# Autodesk Inventor assembly: mg996r_right_mid_top_two_servo
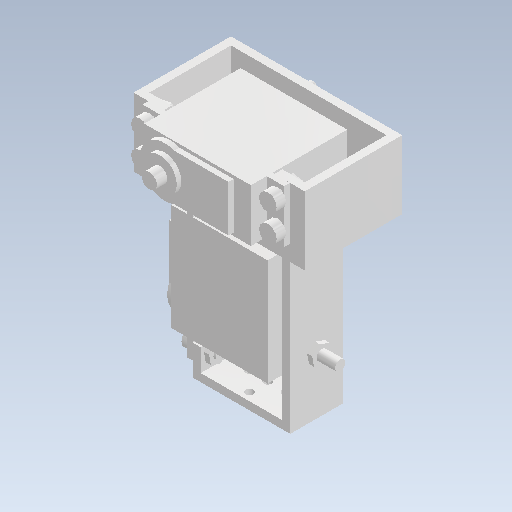
[picture p0: Inventor's stored thumbnail of the model, 512x512]
Saved by Autodesk Inventor 2021.4 (Build 254397000, 397)
## iProperties
Created: 2022-07-25
Part Number: mg996r_right_mid_top_two_servo
Document SubType Name: Assembly
Designer: isamu
Author: isamu
## Documents named in this file (4)
- D:\personal_projects\robot\inventor\2021_matlab_compat _v2\motor_with_frames\mg996r_right_mid_top_two_servo.iam
- D:\personal_projects\robot\inventor\2021_matlab_compat _v2\motor_with_frames\mg996r_bottom.iam
- D:\personal_projects\robot\exports\screws\m3 nuts.ipt
- D:\personal_projects\robot\inventor\2021_matlab_compat _v2\motor_with_frames\mg996r_base_motor_with_axis.iam
## Components (7 placed, 3 different names)
1. mg996r_bottom:1 [sub-assembly] — Mate:1, Mate:2, Mate:3
2. m3 nuts:1 — Insert:3
3. m3 nuts:2 — Insert:5
4. m3 nuts:3 — Insert:2
5. m3 nuts:4 — Insert:4
6. m3 nuts:5 — Insert:1
7. mg996r_base_motor_with_axis:1 [sub-assembly] — Mate:1, Mate:2, Mate:3, Insert:1, Insert:2, Insert:3, Insert:4, Insert:5
## Relationships (8: Insert 5, Mate 3)
- Mate:1: mg996r_bottom:1 ↔ mg996r_base_motor_with_axis:1
- Mate:2: mg996r_bottom:1 ↔ mg996r_base_motor_with_axis:1
- Mate:3: mg996r_bottom:1 ↔ mg996r_base_motor_with_axis:1
- Insert:1: m3 nuts:5 ↔ mg996r_base_motor_with_axis:1
- Insert:2: m3 nuts:3 ↔ mg996r_base_motor_with_axis:1
- Insert:3: m3 nuts:1 ↔ mg996r_base_motor_with_axis:1
- Insert:4: m3 nuts:4 ↔ mg996r_base_motor_with_axis:1
- Insert:5: m3 nuts:2 ↔ mg996r_base_motor_with_axis:1
